# Autodesk Inventor assembly: GimbalFInal
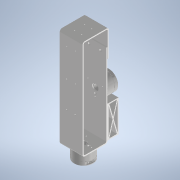
[picture p0: Inventor's stored thumbnail of the model, 180x180]
Saved by Autodesk Inventor 2022 (Build 260153000, 153)
## iProperties
Created: 2023-02-27
Part Number: GimbalFInal
Document SubType Name: Assembly
Designer: mihir
Author: mihir
## Documents named in this file (3)
- C:\Users\mihir\Documents\Personal\InventorBuilds\Room\GimbalFInal.iam
- C:\Users\mihir\Downloads\gimbal.ipt
- C:\Users\mihir\Downloads\FLC 2020 Sentry LG2 march_RoboMaster GM6020 Brushless DC Motor v1 v1.ipt
## Components (3 placed, 2 different names)
1. gimbal:1 — Mate:2, Mate:3, Mate:4, Mate:5
2. FLC 2020 Sentry LG2 march_RoboMaster GM6020 Brushless DC Motor v1 v1:1 — Mate:2, Mate:3
3. FLC 2020 Sentry LG2 march_RoboMaster GM6020 Brushless DC Motor v1 v1:2 — Mate:4, Mate:5
## Relationships (4: Mate 4)
- Mate:2: gimbal:1 ↔ FLC 2020 Sentry LG2 march_RoboMaster GM6020 Brushless DC Motor v1 v1:1
- Mate:3: gimbal:1 ↔ FLC 2020 Sentry LG2 march_RoboMaster GM6020 Brushless DC Motor v1 v1:1
- Mate:4: gimbal:1 ↔ FLC 2020 Sentry LG2 march_RoboMaster GM6020 Brushless DC Motor v1 v1:2
- Mate:5: gimbal:1 ↔ FLC 2020 Sentry LG2 march_RoboMaster GM6020 Brushless DC Motor v1 v1:2
